# Autodesk Inventor assembly: Co_Cau_Truc_Z
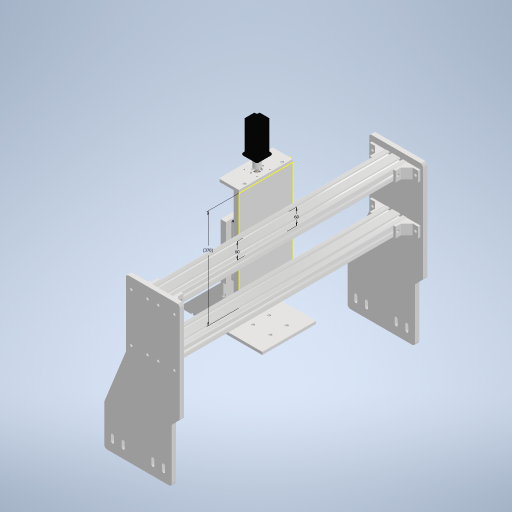
[picture p0: Inventor's stored thumbnail of the model, 512x512]
Saved by Autodesk Inventor 2023 (Build 270158000, 158)
## iProperties
Created: 2025-04-17
Part Number: Co_Cau_Truc_Z
Document SubType Name: Assembly
Designer: huyqu
Author: huyqu
## Documents named in this file (7)
- E:\TAI LIEU\Final_Project\DONE\CoCauTrucZ\Co_Cau_Truc_Z.iam
- E:\TAI LIEU\Final_Project\DONE\CoCauTrucZ\Part_dung.iam
- E:\TAI LIEU\Final_Project\DONE\CoCauTrucZ\Truc_Z.iam
- E:\TAI LIEU\Final_Project\DONE\CoCauTrucZ\Ban_Truot.ipt
- E:\TAI LIEU\Final_Project\DONE\CoCauTrucZ\Part_Truot_T_Nhom.iam
- E:\TAI LIEU\Final_Project\DONE\CoCauTrucZ\Nema23.ipt
- E:\TAI LIEU\Final_Project\DONE\CoCauTrucZ\Khop_noi_mem.ipt
## Components (6 placed, 6 different names)
1. Part_dung:1 [sub-assembly] — Mate:1, Mate:2, Flush:1
2. Truc_Z:1 [sub-assembly] — Mate:1, Mate:2, Flush:1, Mate:3, Mate:4, Mate:5, Mate:9, Mate:10, Mate:12
3. Ban_Truot:1 — Mate:3, Mate:4, Mate:5, Mate:6, Mate:7, Mate:8
4. Part_Truot_T_Nhom:1 [sub-assembly] — Mate:6, Mate:7, Mate:8
5. Nema23:1 — Mate:11, Mate:12
6. Khop_noi_mem:1 — Mate:9, Mate:10, Mate:11
## Relationships (13: Mate 12, Flush 1)
- Mate:1: Part_dung:1 ↔ Truc_Z:1
- Mate:2 (344 mm): Part_dung:1 ↔ Truc_Z:1
- Flush:1 (-30 mm): Part_dung:1 ↔ Truc_Z:1
- Mate:3: Truc_Z:1 ↔ Ban_Truot:1
- Mate:4: Truc_Z:1 ↔ Ban_Truot:1
- Mate:5: Truc_Z:1 ↔ Ban_Truot:1
- Mate:6: Ban_Truot:1 ↔ Part_Truot_T_Nhom:1
- Mate:7: Ban_Truot:1 ↔ Part_Truot_T_Nhom:1
- Mate:8: Ban_Truot:1 ↔ Part_Truot_T_Nhom:1
- Mate:9: Truc_Z:1 ↔ Khop_noi_mem:1
- Mate:10 (8 mm): Truc_Z:1 ↔ Khop_noi_mem:1
- Mate:11: Nema23:1 ↔ Khop_noi_mem:1
- Mate:12: Truc_Z:1 ↔ Nema23:1
